# Autodesk Inventor assembly: 1stLayout
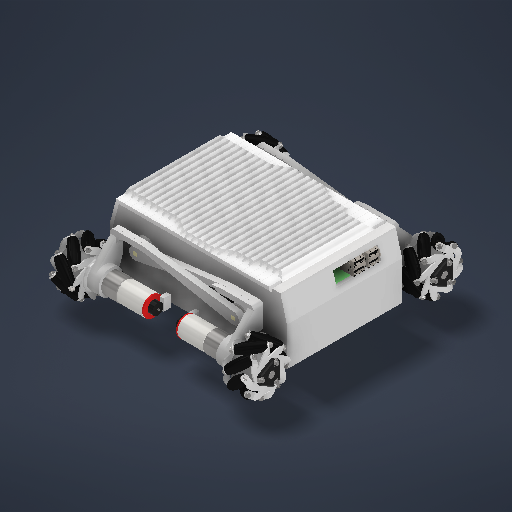
[picture p0: Inventor's stored thumbnail of the model, 512x512]
Saved by Autodesk Inventor 2025 (Build 290162000, 162)
## iProperties
Created: 2024-10-02
Part Number: 1stLayout
Document SubType Name: Assembly
Designer: khrip
Author: khrip
## Documents named in this file (21)
- H:\Potamon\3Dmodels\Chassis\1stLayout.iam
- H:\Potamon\3Dmodels\UnsprungUnits\Wheels\wheel assembly.iam
- H:\Potamon\3Dmodels\UnsprungUnits\Wheels\wheel assemblyMirrored.iam
- H:\Potamon\3Dmodels\UnsprungUnits\Parts\servo.ipt
- H:\Potamon\3Dmodels\Chassis\MaxDimensions.ipt
- H:\Potamon\3Dmodels\Chassis\Parts\ServocontrollerSizer.ipt
- H:\Potamon\3Dmodels\Parts\raspberry\RaspberryPi2 STEP214.iam
- H:\Potamon\3Dmodels\Parts\18650_X6\18650_X6.ipt
- C:\Users\khrip\Documents\Inventor\Content Center Files\R2025\ru-RU\JIS B 1521\JIS B 1521 - 6801 12x21x5x1,92.ipt
- H:\Potamon\3Dmodels\UnsprungUnits\Parts\Knuckle.ipt
- C:\Users\khrip\Documents\Inventor\Content Center Files\R2025\ru-RU\JIS B 1521\JIS B 1521 - 698 8x19x6x2,24.ipt
- H:\Potamon\3Dmodels\SusUnit\Torsion.ipt
- H:\Potamon\3Dmodels\SusUnit\Arm.ipt
- H:\Potamon\3Dmodels\SusUnit\Arm_MIR.ipt
- H:\Potamon\3Dmodels\UnsprungUnits\Parts\Knuckle_MIR.ipt
- H:\Potamon\3Dmodels\UnsprungUnits\Parts\Knuckle_MIR1.ipt
- H:\Potamon\3Dmodels\UnsprungUnits\Parts\Knuckle_MIR_MIR.ipt
- H:\Potamon\3Dmodels\SusUnit\body.ipt
- H:\Potamon\3Dmodels\SusUnit\hood.ipt
- H:\Potamon\3Dmodels\SusUnit\BUMPER.ipt
- H:\Potamon\3Dmodels\SusUnit\BUMPER_MIR.ipt
## Components (37 placed, 20 different names)
1. wheel assembly:1 [sub-assembly] — Заподлицо:2, Совмещение:1, Заподлицо:3, Совмещение:10, Совмещение:15, Совмещение:21, Совмещение:22
2. wheel assemblyMirrored:1 [sub-assembly] — Заподлицо:1, Совмещение:2, Заподлицо:4, Совмещение:9, Совмещение:14, Совмещение:19, Совмещение:20
3. wheel assembly:2 [sub-assembly] — Совмещение:4, Совмещение:5, Совмещение:8, Совмещение:12, Совмещение:13, Совмещение:17, Совмещение:18, Заподлицо:6
4. wheel assemblyMirrored:2 [sub-assembly] — Совмещение:3, Совмещение:6, Совмещение:7, Совмещение:11, Совмещение:16, Совмещение:23, Совмещение:24
5. servo:1 — Угол:1, Совмещение:9, Совмещение:14
6. servo:2 — Угол:2, Совмещение:10, Совмещение:15
7. servo:3 — Угол:3, Совмещение:11, Совмещение:16
8. servo:4 — Угол:4, Совмещение:12, Совмещение:13, Заподлицо:7
9. MaxDimensions:1 — Заподлицо:5
10. ServocontrollerSizer:1
11. ServocontrollerSizer:2
12. RaspberryPi2 STEP214:1 [sub-assembly]
13. 18650_X6:1 — Угол:5, Угол:6
14. JIS B 1521 6801 12x21x5:1 — Совмещение:17, Совмещение:18
15. JIS B 1521 6801 12x21x5:2 — Совмещение:19, Совмещение:20
16. JIS B 1521 6801 12x21x5:3 — Совмещение:21, Совмещение:22
17. JIS B 1521 6801 12x21x5:4 — Совмещение:23, Совмещение:24
18. Knuckle:1 — Заподлицо:6, Заподлицо:7, Заподлицо:8, Совмещение:25, Совмещение:26, Совмещение:27, Совмещение:28, Угол:9, Угол:10, Заподлицо:12, Заподлицо:13
19. JIS B 1521 698 8x19x6:1 — Совмещение:25, Совмещение:26, Заподлицо:10, Совмещение:32, Совмещение:35
20. JIS B 1521 698 8x19x6:2 — Совмещение:27, Совмещение:28, Заподлицо:9, Совмещение:29
21. Torsion:1 — Заподлицо:9, Совмещение:30, Заподлицо:11, Совмещение:31
22. Torsion:2 — Заподлицо:10, Совмещение:33, Совмещение:34
23. Arm:1 — Совмещение:29, Совмещение:30, Заподлицо:11, Совмещение:31, Угол:9, Совмещение:37, Заподлицо:13
24. Arm_MIR:1 — Совмещение:32, Совмещение:33, Совмещение:34, Совмещение:35, Угол:10, Совмещение:37, Заподлицо:12
25. Knuckle_MIR:1 — Совмещение:36
26. Knuckle_MIR1:1 — Совмещение:38, Совмещение:39, Совмещение:40, Совмещение:41, Совмещение:42, Совмещение:43, Угол:11, Совмещение:47, Угол:12
27. JIS B 1521 698 8x19x6:3 — Совмещение:39, Совмещение:40, Заподлицо:15, Совмещение:49, Совмещение:52
28. JIS B 1521 698 8x19x6:4 — Совмещение:41, Совмещение:42, Заподлицо:14, Совмещение:46
29. Torsion:3 — Заподлицо:14, Совмещение:44, Заподлицо:16, Совмещение:45
30. Torsion:4 — Заподлицо:15, Совмещение:50, Совмещение:51
31. Arm:2 — Совмещение:43, Угол:11, Совмещение:44, Заподлицо:16, Совмещение:45, Совмещение:46, Совмещение:48
32. Arm_MIR:2 — Совмещение:47, Совмещение:48, Угол:12, Совмещение:49, Совмещение:50, Совмещение:51, Совмещение:52
33. Knuckle_MIR_MIR:1 — Заподлицо:17
34. body:1 — Заподлицо:18, Заподлицо:19, Совмещение:53, Заподлицо:20, Заподлицо:21, Заподлицо:22, Заподлицо:23
35. hood:1 — Заподлицо:19, Совмещение:53, Заподлицо:20
36. BUMPER:1 — Заподлицо:21, Заподлицо:22, Заподлицо:23
37. BUMPER_MIR:1
## Relationships (86: Mate 53, Flush 23, Angle 10)
- Заподлицо:1 [Flush] (105 mm): wheel assemblyMirrored:1
- Заподлицо:2 [Flush] (105 mm): wheel assembly:1
- Совмещение:1 [Mate] (30 mm): wheel assembly:1
- Совмещение:2 [Mate] (30 mm): wheel assemblyMirrored:1
- Заподлицо:3 [Flush] (105 mm): wheel assembly:1
- Заподлицо:4 [Flush] (-105 mm): wheel assemblyMirrored:1
- Совмещение:3 [Mate] (105 mm): wheel assemblyMirrored:2
- Совмещение:4 [Mate] (105 mm): wheel assembly:2
- Совмещение:5 [Mate] (30 mm): wheel assembly:2
- Совмещение:6 [Mate] (30 mm): wheel assemblyMirrored:2
- Совмещение:7 [Mate] (-105 mm): wheel assemblyMirrored:2
- Совмещение:8 [Mate] (105 mm): wheel assembly:2
- Угол:1 [Angle] (180 deg): servo:1
- Совмещение:9 [Mate]: wheel assemblyMirrored:1 ↔ servo:1
- Угол:2 [Angle] (0 deg): servo:2
- Совмещение:10 [Mate]: wheel assembly:1 ↔ servo:2
- Угол:3 [Angle] (0 deg): servo:3
- Совмещение:11 [Mate]: wheel assemblyMirrored:2 ↔ servo:3
- Угол:4 [Angle] (180 deg): servo:4
- Совмещение:12 [Mate]: wheel assembly:2 ↔ servo:4
- Заподлицо:5 [Flush]: MaxDimensions:1
- Угол:5 [Angle] (180 deg): 18650_X6:1
- Угол:6 [Angle] (0 deg): 18650_X6:1
- Совмещение:13 [Mate] (0.5 mm): wheel assembly:2 ↔ servo:4
- Совмещение:14 [Mate] (0.5 mm): wheel assemblyMirrored:1 ↔ servo:1
- Совмещение:15 [Mate] (0.5 mm): wheel assembly:1 ↔ servo:2
- Совмещение:16 [Mate] (0.5 mm): wheel assemblyMirrored:2 ↔ servo:3
- Совмещение:17 [Mate]: wheel assembly:2 ↔ JIS B 1521 6801 12x21x5:1
- Совмещение:18 [Mate]: wheel assembly:2 ↔ JIS B 1521 6801 12x21x5:1
- Совмещение:19 [Mate]: wheel assemblyMirrored:1 ↔ JIS B 1521 6801 12x21x5:2
- Совмещение:20 [Mate]: wheel assemblyMirrored:1 ↔ JIS B 1521 6801 12x21x5:2
- Совмещение:21 [Mate]: wheel assembly:1 ↔ JIS B 1521 6801 12x21x5:3
- Совмещение:22 [Mate]: wheel assembly:1 ↔ JIS B 1521 6801 12x21x5:3
- Совмещение:23 [Mate]: wheel assemblyMirrored:2 ↔ JIS B 1521 6801 12x21x5:4
- Совмещение:24 [Mate]: wheel assemblyMirrored:2 ↔ JIS B 1521 6801 12x21x5:4
- Заподлицо:6 [Flush]: wheel assembly:2 ↔ Knuckle:1
- Заподлицо:7 [Flush]: servo:4 ↔ Knuckle:1
- Заподлицо:8 [Flush]: Knuckle:1
- Совмещение:25 [Mate] (63.88 mm): Knuckle:1 ↔ JIS B 1521 698 8x19x6:1
- Совмещение:26 [Mate] (52.82 mm): Knuckle:1 ↔ JIS B 1521 698 8x19x6:1
- Совмещение:27 [Mate] (-63.88 mm): Knuckle:1 ↔ JIS B 1521 698 8x19x6:2
- Совмещение:28 [Mate] (52.82 mm): Knuckle:1 ↔ JIS B 1521 698 8x19x6:2
- Заподлицо:9 [Flush] (-7 mm): JIS B 1521 698 8x19x6:2 ↔ Torsion:1
- Заподлицо:10 [Flush] (-7 mm): JIS B 1521 698 8x19x6:1 ↔ Torsion:2
- Совмещение:29 [Mate]: JIS B 1521 698 8x19x6:2 ↔ Arm:1
- Совмещение:30 [Mate]: Torsion:1 ↔ Arm:1
- Заподлицо:11 [Flush]: Torsion:1 ↔ Arm:1
- Совмещение:31 [Mate]: Torsion:1 ↔ Arm:1
- Угол:9 [Angle] (0 deg): Knuckle:1 ↔ Arm:1
- Совмещение:32 [Mate]: JIS B 1521 698 8x19x6:1 ↔ Arm_MIR:1
- Совмещение:33 [Mate]: Torsion:2 ↔ Arm_MIR:1
- Совмещение:34 [Mate]: Torsion:2 ↔ Arm_MIR:1
- Совмещение:35 [Mate]: JIS B 1521 698 8x19x6:1 ↔ Arm_MIR:1
- Угол:10 [Angle] (0 deg): Knuckle:1 ↔ Arm_MIR:1
- Совмещение:36 [Mate]: Knuckle_MIR:1
- Совмещение:37 [Mate] (1 mm): Arm:1 ↔ Arm_MIR:1
- Заподлицо:12 [Flush] (13.5 mm): Knuckle:1 ↔ Arm_MIR:1
- Заподлицо:13 [Flush]: Knuckle:1 ↔ Arm:1
- Совмещение:38 [Mate]: Knuckle_MIR1:1
- Совмещение:39 [Mate] (-52.82 mm): Knuckle_MIR1:1 ↔ JIS B 1521 698 8x19x6:3
- Совмещение:40 [Mate] (-63.88 mm): Knuckle_MIR1:1 ↔ JIS B 1521 698 8x19x6:3
- Совмещение:41 [Mate] (-52.82 mm): Knuckle_MIR1:1 ↔ JIS B 1521 698 8x19x6:4
- Совмещение:42 [Mate] (63.88 mm): Knuckle_MIR1:1 ↔ JIS B 1521 698 8x19x6:4
- Заподлицо:14 [Flush] (-7 mm): JIS B 1521 698 8x19x6:4 ↔ Torsion:3
- Заподлицо:15 [Flush] (-7 mm): JIS B 1521 698 8x19x6:3 ↔ Torsion:4
- Совмещение:43 [Mate]: Knuckle_MIR1:1 ↔ Arm:2
- Угол:11 [Angle] (0 deg): Knuckle_MIR1:1 ↔ Arm:2
- Совмещение:44 [Mate]: Torsion:3 ↔ Arm:2
- Заподлицо:16 [Flush]: Torsion:3 ↔ Arm:2
- Совмещение:45 [Mate]: Torsion:3 ↔ Arm:2
- Совмещение:46 [Mate]: JIS B 1521 698 8x19x6:4 ↔ Arm:2
- Совмещение:47 [Mate] (13.5 mm): Knuckle_MIR1:1 ↔ Arm_MIR:2
- Совмещение:48 [Mate] (1 mm): Arm:2 ↔ Arm_MIR:2
- Угол:12 [Angle] (0 deg): Knuckle_MIR1:1 ↔ Arm_MIR:2
- Совмещение:49 [Mate]: JIS B 1521 698 8x19x6:3 ↔ Arm_MIR:2
- Совмещение:50 [Mate]: Torsion:4 ↔ Arm_MIR:2
- Совмещение:51 [Mate]: Torsion:4 ↔ Arm_MIR:2
- Совмещение:52 [Mate]: JIS B 1521 698 8x19x6:3 ↔ Arm_MIR:2
- Заподлицо:17 [Flush]: Knuckle_MIR_MIR:1
- Заподлицо:18 [Flush]: body:1
- Заподлицо:19 [Flush]: body:1 ↔ hood:1
- Совмещение:53 [Mate] (15 mm): body:1 ↔ hood:1
- Заподлицо:20 [Flush] (10 mm): body:1 ↔ hood:1
- Заподлицо:21 [Flush]: body:1 ↔ BUMPER:1
- Заподлицо:22 [Flush]: body:1 ↔ BUMPER:1
- Заподлицо:23 [Flush]: body:1 ↔ BUMPER:1
